# Autodesk Inventor assembly: Tank Tread Assembly
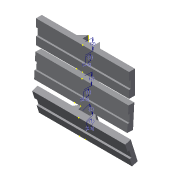
[picture p0: Inventor's stored thumbnail of the model, 180x180]
Saved by Autodesk Inventor 2015 (Build 190159000, 159)
## iProperties
Created: 2015-03-14
Part Number: Tank Tread Assembly
Document SubType Name: Assembly
Designer: james_000
Author: james_000
## Documents named in this file (3)
- C:\Users\james_000\Documents\Inventor\Test\Tank Tread Assembly.iam
- C:\Users\james_000\Documents\Inventor\Test\Tank Tread link A.ipt
- C:\Users\james_000\Documents\Inventor\Test\Tank Tread link B.ipt
## Components (5 placed, 2 different names)
1. Tank Tread link A:1 — Rotational:2, Rotational:3
2. Tank Tread link A:2 — Rotational:1
3. Tank Tread link B:1 — Rotational:1, Rotational:2
4. Tank Tread link B:2 — Rotational:3, Rotational:4
5. Tank Tread link A:3 — Rotational:4
## Relationships (4: RevoluteJoint 4)
- Rotational:1 [RevoluteJoint]: Tank Tread link A:2 ↔ Tank Tread link B:1
- Rotational:2 [RevoluteJoint]: Tank Tread link A:1 ↔ Tank Tread link B:1
- Rotational:3 [RevoluteJoint]: Tank Tread link A:1 ↔ Tank Tread link B:2
- Rotational:4 [RevoluteJoint]: Tank Tread link B:2 ↔ Tank Tread link A:3
